# Autodesk Inventor assembly: Assembly4
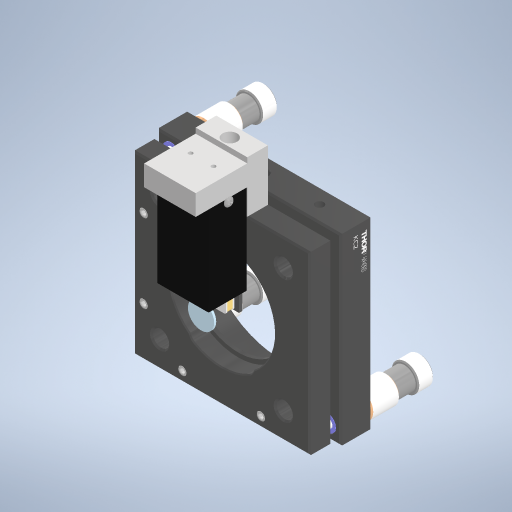
[picture p0: Inventor's stored thumbnail of the model, 512x512]
Saved by Autodesk Inventor 2023 (Build 270158000, 158)
## iProperties
Created: 2024-01-12
Part Number: Assembly4
Document SubType Name: Assembly
Designer: kerlin
Author: kerlin
## Documents named in this file (5)
- C:\Users\kerlin\Documents\KerlinLab\KTN\Multipass\MechanicalDrawing\Assembly4.iam
- C:\Users\kerlin\Downloads\KC2-Solidworks.ipt
- C:\Users\kerlin\Downloads\sc30.ipt
- C:\Users\kerlin\Documents\KerlinLab\KTN\Multipass\MechanicalDrawing\ResonantAdapter.ipt
- C:\Users\kerlin\Documents\KerlinLab\KTN\Multipass\MechanicalDrawing\ResonantSlider.ipt
## Components (4 placed, 4 different names)
1. KC2-Solidworks:1 — Mate:1, Mate:2, Mate:3, Mate:4
2. sc30:1 — Mate:1, Mate:2, Mate:6
3. ResonantAdapter:1 — Mate:3, Mate:4, Mate:5
4. ResonantSlider:1 — Mate:5, Mate:6
## Relationships (6: Mate 6)
- Mate:1: KC2-Solidworks:1 ↔ sc30:1
- Mate:2: KC2-Solidworks:1 ↔ sc30:1
- Mate:3: KC2-Solidworks:1 ↔ ResonantAdapter:1
- Mate:4: KC2-Solidworks:1 ↔ ResonantAdapter:1
- Mate:5: ResonantAdapter:1 ↔ ResonantSlider:1
- Mate:6: sc30:1 ↔ ResonantSlider:1
